# Autodesk Inventor assembly: CNC Router
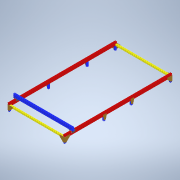
[picture p0: Inventor's stored thumbnail of the model, 180x180]
Saved by Autodesk Inventor 2022.2 (Build 262287010, 287A)
## iProperties
Created: 2022-03-31
Part Number: CNC Router
Document SubType Name: Assembly
Designer: Robert Nies
Author: Robert Nies
## Documents named in this file (3)
- C:\Users\rober\PycharmProjects\CNCRouter\Master Assembly\CNC Router.iam
- C:\Users\rober\PycharmProjects\CNCRouter\Master Assembly\Frame\Frame.iam
- C:\Users\rober\PycharmProjects\CNCRouter\Master Assembly\Gantry\Gantry.iam
## Components (2 placed, 2 different names)
1. Frame:1 [sub-assembly] — Mate:3, Mate:4
2. Gantry:1 [sub-assembly] — Mate:3, Mate:4
## Relationships (2: Mate 2)
- Mate:3: Frame:1 ↔ Gantry:1
- Mate:4: Frame:1 ↔ Gantry:1
